# Autodesk Inventor assembly: Finger Assembly
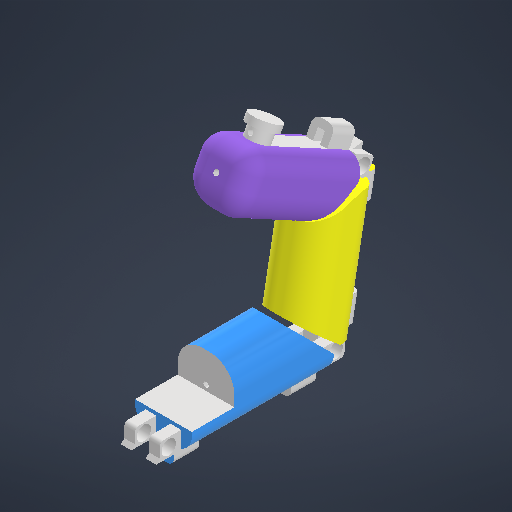
[picture p0: Inventor's stored thumbnail of the model, 512x512]
Saved by Autodesk Inventor 2026 (Build 300175050, 175E)
## iProperties
Created: 2026-05-23
Part Number: Finger Assembly
Document SubType Name: Assembly
Designer: SaiAn
Author: SaiAn
## Documents named in this file (4)
- C:\EMG Biomechanical Arm\Finger Assembly.iam
- C:\EMG Biomechanical Arm\FingerMiddle.ipt
- C:\EMG Biomechanical Arm\FingerTop.ipt
- C:\EMG Biomechanical Arm\FingerBase.ipt
## Components (3 placed, 3 different names)
1. FingerTop:1 — Mate:1, Mate:2, Mate:3
2. FingerMiddle:1 — Mate:1, Mate:2, Mate:3, Mate:4, Mate:5
3. FingerBase:1 — Mate:4, Mate:5
## Relationships (5: Mate 5)
- Mate:1: FingerTop:1 ↔ FingerMiddle:1
- Mate:2: FingerTop:1 ↔ FingerMiddle:1
- Mate:3: FingerTop:1 ↔ FingerMiddle:1
- Mate:4: FingerMiddle:1 ↔ FingerBase:1
- Mate:5: FingerMiddle:1 ↔ FingerBase:1
